# Autodesk Inventor assembly: mikrosumo
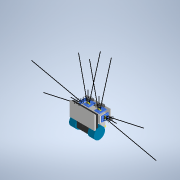
[picture p0: Inventor's stored thumbnail of the model, 180x180]
Saved by Autodesk Inventor 2022 (Build 260153000, 153)
## iProperties
Created: 2022-12-13
Part Number: mikrosumo
Document SubType Name: Assembly
Designer: komputer
Author: komputer
## Documents named in this file (10)
- D:\Inventor\MikroSumo\mikrosumo.iam
- D:\Inventor\MikroSumo\podsta.ipt
- D:\Inventor\MikroSumo\koło.ipt
- D:\Inventor\MikroSumo\opona.ipt
- D:\Inventor\MikroSumo\pokrywa silników.ipt
- D:\Inventor\MikroSumo\lipol 150mAH.ipt
- D:\Inventor\MikroSumo\nozz.ipt
- C:\Users\Kamil\Desktop\pulpit\powerhd_hd_1370a_micro.ipt
- D:\KONARM\konarm 3 przegub\pcbek.ipt
- C:\Users\Kamil\Desktop\TOF_VLCOS.ipt
## Components (15 placed, 9 different names)
1. podsta:1 — Flush:1, Mate:1, Flush:2
2. koło:1
3. koło:2
4. opona:1
5. opona:2
6. lipol 150mAH:1
7. nozz:1
8. pokrywa silników:2 — Flush:1, Mate:1, Flush:2, Flush:6, Mate:3
9. pcbek:1 — Flush:6, Mate:2, Mate:4, Mate:5, Mate:6, Mate:7, Mate:8, Flush:8, Mate:9, Mate:11, Mate:12, Mate:14, Flush:9
10. powerhd_hd_1370a_micro:1 — Mate:2, Mate:3, Mate:4, Flush:7
11. powerhd_hd_1370a_micro:2 — Mate:5, Mate:6, Flush:7
12. TOF_VLCOS:1 — Mate:7, Mate:11, Mate:16
13. TOF_VLCOS:2 — Mate:8, Flush:8, Mate:12, Mate:16, Flush:10
14. TOF_VLCOS:3 — Mate:9, Mate:14
15. TOF_VLCOS:5 — Flush:9, Flush:10
## Relationships (20: Mate 13, Flush 7)
- Flush:1: podsta:1 ↔ pokrywa silników:2
- Mate:1 (11.5 mm): podsta:1 ↔ pokrywa silników:2
- Flush:2: podsta:1 ↔ pokrywa silników:2
- Flush:6: pokrywa silników:2 ↔ pcbek:1
- Mate:2: pcbek:1 ↔ powerhd_hd_1370a_micro:1
- Mate:3: pokrywa silników:2 ↔ powerhd_hd_1370a_micro:1
- Mate:4: pcbek:1 ↔ powerhd_hd_1370a_micro:1
- Mate:5: pcbek:1 ↔ powerhd_hd_1370a_micro:2
- Mate:6: pcbek:1 ↔ powerhd_hd_1370a_micro:2
- Flush:7: powerhd_hd_1370a_micro:1 ↔ powerhd_hd_1370a_micro:2
- Mate:7 (-4 mm): pcbek:1 ↔ TOF_VLCOS:1
- Mate:8 (-4 mm): pcbek:1 ↔ TOF_VLCOS:2
- Flush:8 (2 mm): pcbek:1 ↔ TOF_VLCOS:2
- Mate:9 (-4 mm): pcbek:1 ↔ TOF_VLCOS:3
- Mate:11: pcbek:1 ↔ TOF_VLCOS:1
- Mate:12: pcbek:1 ↔ TOF_VLCOS:2
- Mate:14: pcbek:1 ↔ TOF_VLCOS:3
- Mate:16 (7.8 mm): TOF_VLCOS:1 ↔ TOF_VLCOS:2
- Flush:9 (-2.4 mm): pcbek:1 ↔ TOF_VLCOS:5
- Flush:10: TOF_VLCOS:2 ↔ TOF_VLCOS:5
